# Autodesk Inventor assembly: ASY PRS 2 Filter column D1200
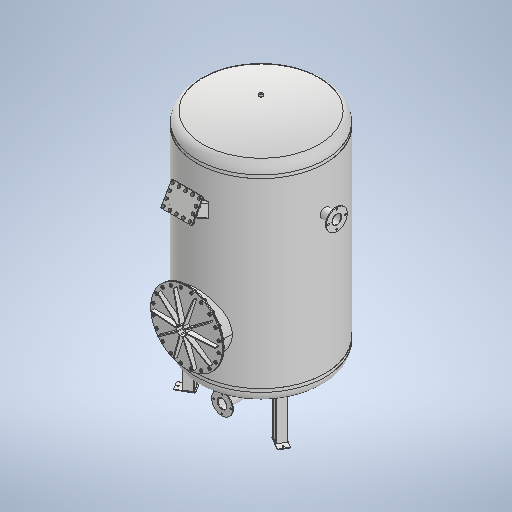
[picture p0: Inventor's stored thumbnail of the model, 512x512]
Saved by Autodesk Inventor 2026.2 (Build 302298000, 298)
## iProperties
Created: 2025-02-13
Part Number: ASY PRS 2 Filter column D1200
Document SubType Name: Assembly
Designer: admin
Mass: 296006 g
Surface Area: 199460 cm^2
Volume: 66339.5 cm^3
Density: 4.46198 g/cm^3
Author: pokla
Revision Number: 3
## Documents named in this file (23)
- C:\Users\admin\Documents\Inventor\PRS-Purovsk\ASY PRS 2 Filter column D1200.iam
- C:\Users\admin\Documents\Inventor\PRS-Purovsk\PRS 0101 main shell D1200.ipt
- C:\Users\admin\Documents\Inventor\PRS-Purovsk\PRS 1604 dished head_D1200.ipt
- C:\Users\admin\Documents\Inventor\PRS-Purovsk\Fitting G1_D1200.ipt
- C:\Users\admin\Documents\Inventor\PRS-Purovsk\PRS 1633 charging blind flange_D1200.ipt
- C:\Users\admin\Documents\Inventor\PRS-Purovsk\ASY PRS 1791 top funnel 50-90_1000x90_D1200.iam
- C:\Users\admin\Documents\Inventor\PRS-Purovsk\PRS 8123 pallet jack dummy_D1200.ipt
- C:\Users\admin\Documents\Inventor\PRS-Purovsk\ASY PRS 1610 charging hatch_D1200.iam
- C:\Users\admin\Documents\Inventor\PRS-Purovsk\PRS 9612 accses hatch flangeipt_D1200.ipt
- C:\Users\admin\Documents\Inventor\PRS-Purovsk\PRS 9615 FDS tube 5_D1200.ipt
- C:\Users\admin\Documents\Inventor\PRS-Purovsk\PRS 9612 FDS tube 2_D1200.ipt
- C:\Users\admin\Documents\Inventor\PRS-Purovsk\cc\JIS B 2312 90 Deg Long Elbow Steel 80A x Sch 40.ipt
- C:\Users\admin\Documents\Inventor\PRS-Purovsk\PRS 9311 accses hatch tube_D1200.ipt
- C:\Users\admin\Documents\Inventor\PRS-Purovsk\PRS 9432 FDS free flange DN90_D1200.ipt
- C:\Users\admin\Documents\Inventor\PRS-Purovsk\PRS 9431 FDS flange DN90_D1200.ipt
- C:\Users\admin\Documents\Inventor\PRS-Purovsk\PRS 9614 FDS tube 4_D1200.ipt
- C:\Users\admin\Documents\Inventor\PRS-Purovsk\PRS 9613 FDS tube 3_D1200.ipt
- C:\Users\admin\Documents\Inventor\PRS-Purovsk\ASY PRS 9690 Filter legs D1200.iam
- C:\Users\admin\Documents\Inventor\PRS-Purovsk\ASY PRS 9800 DrainSystemBottom_D1200.iam
- C:\Users\admin\Documents\Inventor\PRS-Purovsk\cc\en-US\ISO 4018\ISO 4018 - M16 x 40.ipt
- C:\Users\admin\Documents\Inventor\PRS-Purovsk\cc\en-US\ISO 7089\ISO 7089 - 16 - 140 HV(1).ipt
- C:\Users\admin\Documents\Inventor\PRS-Purovsk\cc\en-US\ISO 4032(2)\ISO 4032 - M16 - ISO.ipt
- C:\Users\admin\Documents\Inventor\PRS-Purovsk\ASY 9610 charging hatch.iam
## Components (84 placed, 22 different names)
1. PRS 0101 main shell D1200:1 — Flush:2, Rigid:14, Rigid:15, Rigid:16, Flush:4, Mate:1, Mate:3
2. PRS 1604 dished head_D1200:1 — Rigid:15, Mate:5, Rigid:20, Mate:8
3. PRS 1604 dished head_D1200:2 — Rigid:15, Rigid:14, Mate:4
4. Fitting G1_D1200:1 — Rigid:15
5. PRS 1633 charging blind flange_D1200:1 — Rigid:67
6. ASY PRS 1791 top funnel 50-90_1000x90_D1200:1 [sub-assembly] — Rotational:72
7. pallet jack dummy_1200:1
8. PRS 1633 charging blind flange_D1200:2 — Rigid:77
9. PRS 1633 charging blind flange_D1200:3 — Rotational:72, Rigid:78
10. ASY PRS 1610 charging hatch_D1200:1 [sub-assembly] — Rigid:24, Mate:11, Mate:12, Mate:13, Mate:14, Mate:15, Mate:16, Mate:17, Mate:18, Mate:19, Mate:20, Mate:21, Mate:22, Mate:23, Mate:24, Mate:25, Mate:26, Mate:27, Mate:28, Mate:29, Mate:30, Mate:31, Mate:32, Mate:33, Mate:34, Mate:35, Mate:36, Mate:37, Mate:38, Mate:39, Mate:40, Mate:41, Mate:42, Mate:43, Mate:44, Mate:45, Mate:46, Mate:47, Mate:48, Mate:49, Mate:50, Mate:51, Mate:53, Mate:55, Mate:57, Mate:59, Mate:61, Mate:63, Mate:65, Mate:67, Mate:69, Mate:71, Mate:73, Mate:75, Mate:77, Mate:79, Mate:81, Mate:83, Mate:85, Mate:87, Mate:89
11. PRS 9612 accses hatch flangeipt_D1200:1 — Rigid:23, Rigid:24, Mate:52, Mate:54, Mate:56, Mate:58, Mate:60, Mate:62, Mate:64, Mate:66, Mate:68, Mate:70, Mate:72, Mate:74, Mate:76, Mate:78, Mate:80, Mate:82, Mate:84, Mate:86, Mate:88, Mate:90
12. PRS 9615 FDS tube 5_D1200:1 — Rigid:73, Rigid:77, Mate:3
13. PRS 9612 FDS tube 2_D1200:1 — Rigid:62, Rigid:78, Mate:4
14. JIS B 2312 90 Deg Long Elbow Steel 80A x Sch 40:1 — Rigid:62, Rigid:73
15. PRS 9311 accses hatch tube_D1200:1 — Rigid:16, Rigid:23
16. PRS 9432 FDS free flange DN90_D1200:1 — Rigid:76, Rotational:71, Rotational:78
17. PRS 9431 FDS flange DN90_D1200:1 — Rigid:76
18. PRS 9614 FDS tube 4_D1200:1 — Rigid:79, Rotational:71, Rigid:20
19. PRS 9613 FDS tube 3_D1200:1 — Rigid:68, Rigid:67
20. JIS B 2312 90 Deg Long Elbow Steel 80A x Sch 40:2 — Rigid:68, Rigid:79
21. Fitting G1_D1200:2 — Mate:6, Mate:7, Mate:8
22. ASY PRS 9800 DrainSystemBottom_D1200:1 [sub-assembly] — Rotational:78
23. ASY PRS 9690 Filter legs D1200:1 [sub-assembly] — Flush:5, Flush:6, Mate:2
24. ISO 4018 M16 x 40:1 — Mate:11, Mate:12
25. ISO 7089 16:1 — Mate:51, Mate:52, Insert:1
26. ISO 4032 M16:1 — Insert:1
27. ISO 4018 M16 x 40:2 — Mate:13, Mate:14
28. ISO 4018 M16 x 40:3 — Mate:15, Mate:16
29. ISO 4018 M16 x 40:4 — Mate:17, Mate:18
30. ISO 4018 M16 x 40:5 — Mate:19, Mate:20
31. ISO 4018 M16 x 40:6 — Mate:21, Mate:22
32. ISO 4018 M16 x 40:7 — Mate:23, Mate:24
33. ISO 4018 M16 x 40:8 — Mate:25, Mate:26
34. ISO 4018 M16 x 40:9 — Mate:27, Mate:28
35. ISO 4018 M16 x 40:10 — Mate:29, Mate:30
36. ISO 4018 M16 x 40:11 — Mate:31, Mate:32
37. ISO 4018 M16 x 40:12 — Mate:33, Mate:34
38. ISO 4018 M16 x 40:13 — Mate:35, Mate:36
39. ISO 4018 M16 x 40:14 — Mate:37, Mate:38
40. ISO 4018 M16 x 40:15 — Mate:39, Mate:40
41. ISO 4018 M16 x 40:16 — Mate:41, Mate:42
42. ISO 4018 M16 x 40:17 — Mate:43, Mate:44
43. ISO 4018 M16 x 40:18 — Mate:45, Mate:46
44. ISO 4018 M16 x 40:19 — Mate:47, Mate:48
45. ISO 4018 M16 x 40:20 — Mate:49, Mate:50
46. ISO 7089 16:2 — Mate:53, Mate:54, Insert:2
47. ISO 7089 16:3 — Mate:55, Mate:56, Insert:3
48. ISO 7089 16:4 — Mate:57, Mate:58, Insert:4
49. ISO 7089 16:5 — Mate:59, Mate:60, Insert:5
50. ISO 7089 16:6 — Mate:61, Mate:62, Insert:6
51. ISO 7089 16:7 — Mate:63, Mate:64, Insert:7
52. ISO 7089 16:8 — Mate:65, Mate:66, Insert:8
53. ISO 7089 16:9 — Mate:67, Mate:68, Insert:9
54. ISO 7089 16:10 — Mate:69, Mate:70, Insert:10
55. ISO 7089 16:11 — Mate:71, Mate:72, Insert:11
56. ISO 7089 16:12 — Mate:73, Mate:74, Insert:12
57. ISO 7089 16:13 — Mate:75, Mate:76, Insert:13
58. ISO 7089 16:14 — Mate:77, Mate:78, Insert:14
59. ISO 7089 16:15 — Mate:79, Mate:80, Insert:15
60. ISO 7089 16:16 — Mate:81, Mate:82, Insert:16
61. ISO 7089 16:17 — Mate:83, Mate:84, Insert:17
62. ISO 7089 16:18 — Mate:85, Mate:86, Insert:18
63. ISO 7089 16:19 — Mate:87, Mate:88, Insert:19
64. ISO 7089 16:20 — Mate:89, Mate:90, Insert:20
65. ISO 4032 M16:2 — Insert:2
66. ISO 4032 M16:3 — Insert:3
67. ISO 4032 M16:4 — Insert:4
68. ISO 4032 M16:5 — Insert:5
69. ISO 4032 M16:6 — Insert:6
70. ISO 4032 M16:7 — Insert:7
71. ISO 4032 M16:8 — Insert:8
72. ISO 4032 M16:9 — Insert:9
73. ISO 4032 M16:10 — Insert:10
74. ISO 4032 M16:11 — Insert:11
75. ISO 4032 M16:12 — Insert:12
76. ISO 4032 M16:13 — Insert:13
77. ISO 4032 M16:14 — Insert:14
78. ISO 4032 M16:15 — Insert:15
79. ISO 4032 M16:16 — Insert:16
80. ISO 4032 M16:17 — Insert:17
81. ISO 4032 M16:18 — Insert:18
82. ISO 4032 M16:19 — Insert:19
83. ISO 4032 M16:20 — Insert:20
84. ASY 9610 charging hatch:1 [sub-assembly]
## Relationships (133: Mate 90, Insert 20, WeldJoint 15, Flush 4, RevoluteJoint 3, Tangent 1)
- Rigid:15 [WeldJoint]: PRS 1604 dished head_D1200:2 ↔ Fitting G1_D1200:1
- Rigid:62 [WeldJoint]: PRS 9612 FDS tube 2_D1200:1 ↔ JIS B 2312 90 Deg Long Elbow Steel 80A x Sch 40:1
- Rigid:68 [WeldJoint]: PRS 9613 FDS tube 3_D1200:1 ↔ JIS B 2312 90 Deg Long Elbow Steel 80A x Sch 40:2
- Rigid:67 [WeldJoint]: PRS 1633 charging blind flange_D1200:1 ↔ PRS 9613 FDS tube 3_D1200:1
- Rigid:79 [WeldJoint]: PRS 9614 FDS tube 4_D1200:1 ↔ JIS B 2312 90 Deg Long Elbow Steel 80A x Sch 40:2
- Rigid:73 [WeldJoint]: PRS 9615 FDS tube 5_D1200:1 ↔ JIS B 2312 90 Deg Long Elbow Steel 80A x Sch 40:1
- Rigid:76 [WeldJoint]: PRS 9432 FDS free flange DN90_D1200:1 ↔ PRS 9431 FDS flange DN90_D1200:1
- Rotational:71 [RevoluteJoint]: PRS 9432 FDS free flange DN90_D1200:1 ↔ PRS 9614 FDS tube 4_D1200:1
- Rigid:77 [WeldJoint]: PRS 1633 charging blind flange_D1200:2 ↔ PRS 9615 FDS tube 5_D1200:1
- Rotational:72 [RevoluteJoint]: ASY PRS 1791 top funnel 50-90_1000x90_D1200:1 ↔ PRS 1633 charging blind flange_D1200:3
- Rigid:78 [WeldJoint]: PRS 1633 charging blind flange_D1200:3 ↔ PRS 9612 FDS tube 2_D1200:1
- Rotational:78 [RevoluteJoint]: PRS 9432 FDS free flange DN90_D1200:1 ↔ ASY PRS 9800 DrainSystemBottom_D1200:1
- Flush:2: PRS 0101 main shell D1200:1
- Rigid:14 [WeldJoint]: PRS 0101 main shell D1200:1 ↔ PRS 1604 dished head_D1200:2
- Rigid:15 [WeldJoint]: PRS 0101 main shell D1200:1 ↔ PRS 1604 dished head_D1200:1
- Rigid:16 [WeldJoint] (20 mm): PRS 0101 main shell D1200:1 ↔ PRS 9311 accses hatch tube_D1200:1
- Flush:4: PRS 0101 main shell D1200:1
- Mate:1: PRS 0101 main shell D1200:1
- Flush:5: ASY PRS 9690 Filter legs D1200:1
- Flush:6: ASY PRS 9690 Filter legs D1200:1
- Mate:2: ASY PRS 9690 Filter legs D1200:1
- Mate:3: PRS 0101 main shell D1200:1 ↔ PRS 9615 FDS tube 5_D1200:1
- Mate:4: PRS 1604 dished head_D1200:2 ↔ PRS 9612 FDS tube 2_D1200:1
- Mate:5 (300 mm): PRS 1604 dished head_D1200:1
- Rigid:20 [WeldJoint]: PRS 1604 dished head_D1200:1 ↔ PRS 9614 FDS tube 4_D1200:1
- Mate:6: Fitting G1_D1200:2
- Mate:7 (150 mm): Fitting G1_D1200:2
- Mate:8: PRS 1604 dished head_D1200:1 ↔ Fitting G1_D1200:2
- [Mate]: PRS 0101 main shell D1200:1 ↔ ASY 9610 charging hatch:1
- [Mate]: PRS 0101 main shell D1200:1 ↔ ASY 9610 charging hatch:1
- Rigid:23 [WeldJoint]: PRS 9612 accses hatch flangeipt_D1200:1 ↔ PRS 9311 accses hatch tube_D1200:1
- Rigid:24 [WeldJoint]: ASY PRS 1610 charging hatch_D1200:1 ↔ PRS 9612 accses hatch flangeipt_D1200:1
- [Tangent] (80 mm): PRS 0101 main shell D1200:1 ↔ ASY 9610 charging hatch:1
- Mate:11: ASY PRS 1610 charging hatch_D1200:1 ↔ ISO 4018 M16 x 40:1
- Mate:12: ASY PRS 1610 charging hatch_D1200:1 ↔ ISO 4018 M16 x 40:1
- Mate:13: ASY PRS 1610 charging hatch_D1200:1 ↔ ISO 4018 M16 x 40:2
- Mate:14: ASY PRS 1610 charging hatch_D1200:1 ↔ ISO 4018 M16 x 40:2
- Mate:15: ASY PRS 1610 charging hatch_D1200:1 ↔ ISO 4018 M16 x 40:3
- Mate:16: ASY PRS 1610 charging hatch_D1200:1 ↔ ISO 4018 M16 x 40:3
- Mate:17: ASY PRS 1610 charging hatch_D1200:1 ↔ ISO 4018 M16 x 40:4
- Mate:18: ASY PRS 1610 charging hatch_D1200:1 ↔ ISO 4018 M16 x 40:4
- Mate:19: ASY PRS 1610 charging hatch_D1200:1 ↔ ISO 4018 M16 x 40:5
- Mate:20: ASY PRS 1610 charging hatch_D1200:1 ↔ ISO 4018 M16 x 40:5
- Mate:21: ASY PRS 1610 charging hatch_D1200:1 ↔ ISO 4018 M16 x 40:6
- Mate:22: ASY PRS 1610 charging hatch_D1200:1 ↔ ISO 4018 M16 x 40:6
- Mate:23: ASY PRS 1610 charging hatch_D1200:1 ↔ ISO 4018 M16 x 40:7
- Mate:24: ASY PRS 1610 charging hatch_D1200:1 ↔ ISO 4018 M16 x 40:7
- Mate:25: ASY PRS 1610 charging hatch_D1200:1 ↔ ISO 4018 M16 x 40:8
- Mate:26: ASY PRS 1610 charging hatch_D1200:1 ↔ ISO 4018 M16 x 40:8
- Mate:27: ASY PRS 1610 charging hatch_D1200:1 ↔ ISO 4018 M16 x 40:9
- Mate:28: ASY PRS 1610 charging hatch_D1200:1 ↔ ISO 4018 M16 x 40:9
- Mate:29: ASY PRS 1610 charging hatch_D1200:1 ↔ ISO 4018 M16 x 40:10
- Mate:30: ASY PRS 1610 charging hatch_D1200:1 ↔ ISO 4018 M16 x 40:10
- Mate:31: ASY PRS 1610 charging hatch_D1200:1 ↔ ISO 4018 M16 x 40:11
- Mate:32: ASY PRS 1610 charging hatch_D1200:1 ↔ ISO 4018 M16 x 40:11
- Mate:33: ASY PRS 1610 charging hatch_D1200:1 ↔ ISO 4018 M16 x 40:12
- Mate:34: ASY PRS 1610 charging hatch_D1200:1 ↔ ISO 4018 M16 x 40:12
- Mate:35: ASY PRS 1610 charging hatch_D1200:1 ↔ ISO 4018 M16 x 40:13
- Mate:36: ASY PRS 1610 charging hatch_D1200:1 ↔ ISO 4018 M16 x 40:13
- Mate:37: ASY PRS 1610 charging hatch_D1200:1 ↔ ISO 4018 M16 x 40:14
- Mate:38: ASY PRS 1610 charging hatch_D1200:1 ↔ ISO 4018 M16 x 40:14
- Mate:39: ASY PRS 1610 charging hatch_D1200:1 ↔ ISO 4018 M16 x 40:15
- Mate:40: ASY PRS 1610 charging hatch_D1200:1 ↔ ISO 4018 M16 x 40:15
- Mate:41: ASY PRS 1610 charging hatch_D1200:1 ↔ ISO 4018 M16 x 40:16
- Mate:42: ASY PRS 1610 charging hatch_D1200:1 ↔ ISO 4018 M16 x 40:16
- Mate:43: ASY PRS 1610 charging hatch_D1200:1 ↔ ISO 4018 M16 x 40:17
- Mate:44: ASY PRS 1610 charging hatch_D1200:1 ↔ ISO 4018 M16 x 40:17
- Mate:45: ASY PRS 1610 charging hatch_D1200:1 ↔ ISO 4018 M16 x 40:18
- Mate:46: ASY PRS 1610 charging hatch_D1200:1 ↔ ISO 4018 M16 x 40:18
- Mate:47: ASY PRS 1610 charging hatch_D1200:1 ↔ ISO 4018 M16 x 40:19
- Mate:48: ASY PRS 1610 charging hatch_D1200:1 ↔ ISO 4018 M16 x 40:19
- Mate:49: ASY PRS 1610 charging hatch_D1200:1 ↔ ISO 4018 M16 x 40:20
- Mate:50: ASY PRS 1610 charging hatch_D1200:1 ↔ ISO 4018 M16 x 40:20
- Mate:51: ASY PRS 1610 charging hatch_D1200:1 ↔ ISO 7089 16:1
- Mate:52: PRS 9612 accses hatch flangeipt_D1200:1 ↔ ISO 7089 16:1
- Mate:53: ASY PRS 1610 charging hatch_D1200:1 ↔ ISO 7089 16:2
- Mate:54: PRS 9612 accses hatch flangeipt_D1200:1 ↔ ISO 7089 16:2
- Mate:55: ASY PRS 1610 charging hatch_D1200:1 ↔ ISO 7089 16:3
- Mate:56: PRS 9612 accses hatch flangeipt_D1200:1 ↔ ISO 7089 16:3
- Mate:57: ASY PRS 1610 charging hatch_D1200:1 ↔ ISO 7089 16:4
- Mate:58: PRS 9612 accses hatch flangeipt_D1200:1 ↔ ISO 7089 16:4
- Mate:59: ASY PRS 1610 charging hatch_D1200:1 ↔ ISO 7089 16:5
- Mate:60: PRS 9612 accses hatch flangeipt_D1200:1 ↔ ISO 7089 16:5
- Mate:61: ASY PRS 1610 charging hatch_D1200:1 ↔ ISO 7089 16:6
- Mate:62: PRS 9612 accses hatch flangeipt_D1200:1 ↔ ISO 7089 16:6
- Mate:63: ASY PRS 1610 charging hatch_D1200:1 ↔ ISO 7089 16:7
- Mate:64: PRS 9612 accses hatch flangeipt_D1200:1 ↔ ISO 7089 16:7
- Mate:65: ASY PRS 1610 charging hatch_D1200:1 ↔ ISO 7089 16:8
- Mate:66: PRS 9612 accses hatch flangeipt_D1200:1 ↔ ISO 7089 16:8
- Mate:67: ASY PRS 1610 charging hatch_D1200:1 ↔ ISO 7089 16:9
- Mate:68: PRS 9612 accses hatch flangeipt_D1200:1 ↔ ISO 7089 16:9
- Mate:69: ASY PRS 1610 charging hatch_D1200:1 ↔ ISO 7089 16:10
- Mate:70: PRS 9612 accses hatch flangeipt_D1200:1 ↔ ISO 7089 16:10
- Mate:71: ASY PRS 1610 charging hatch_D1200:1 ↔ ISO 7089 16:11
- Mate:72: PRS 9612 accses hatch flangeipt_D1200:1 ↔ ISO 7089 16:11
- Mate:73: ASY PRS 1610 charging hatch_D1200:1 ↔ ISO 7089 16:12
- Mate:74: PRS 9612 accses hatch flangeipt_D1200:1 ↔ ISO 7089 16:12
- Mate:75: ASY PRS 1610 charging hatch_D1200:1 ↔ ISO 7089 16:13
- Mate:76: PRS 9612 accses hatch flangeipt_D1200:1 ↔ ISO 7089 16:13
- Mate:77: ASY PRS 1610 charging hatch_D1200:1 ↔ ISO 7089 16:14
- Mate:78: PRS 9612 accses hatch flangeipt_D1200:1 ↔ ISO 7089 16:14
- Mate:79: ASY PRS 1610 charging hatch_D1200:1 ↔ ISO 7089 16:15
- Mate:80: PRS 9612 accses hatch flangeipt_D1200:1 ↔ ISO 7089 16:15
- Mate:81: ASY PRS 1610 charging hatch_D1200:1 ↔ ISO 7089 16:16
- Mate:82: PRS 9612 accses hatch flangeipt_D1200:1 ↔ ISO 7089 16:16
- Mate:83: ASY PRS 1610 charging hatch_D1200:1 ↔ ISO 7089 16:17
- Mate:84: PRS 9612 accses hatch flangeipt_D1200:1 ↔ ISO 7089 16:17
- Mate:85: ASY PRS 1610 charging hatch_D1200:1 ↔ ISO 7089 16:18
- Mate:86: PRS 9612 accses hatch flangeipt_D1200:1 ↔ ISO 7089 16:18
- Mate:87: ASY PRS 1610 charging hatch_D1200:1 ↔ ISO 7089 16:19
- Mate:88: PRS 9612 accses hatch flangeipt_D1200:1 ↔ ISO 7089 16:19
- Mate:89: ASY PRS 1610 charging hatch_D1200:1 ↔ ISO 7089 16:20
- Mate:90: PRS 9612 accses hatch flangeipt_D1200:1 ↔ ISO 7089 16:20
- Insert:1: ISO 7089 16:1 ↔ ISO 4032 M16:1
- Insert:2: ISO 7089 16:2 ↔ ISO 4032 M16:2
- Insert:3: ISO 7089 16:3 ↔ ISO 4032 M16:3
- Insert:4: ISO 7089 16:4 ↔ ISO 4032 M16:4
- Insert:5: ISO 7089 16:5 ↔ ISO 4032 M16:5
- Insert:6: ISO 7089 16:6 ↔ ISO 4032 M16:6
- Insert:7: ISO 7089 16:7 ↔ ISO 4032 M16:7
- Insert:8: ISO 7089 16:8 ↔ ISO 4032 M16:8
- Insert:9: ISO 7089 16:9 ↔ ISO 4032 M16:9
- Insert:10: ISO 7089 16:10 ↔ ISO 4032 M16:10
- Insert:11: ISO 7089 16:11 ↔ ISO 4032 M16:11
- Insert:12: ISO 7089 16:12 ↔ ISO 4032 M16:12
- Insert:13: ISO 7089 16:13 ↔ ISO 4032 M16:13
- Insert:14: ISO 7089 16:14 ↔ ISO 4032 M16:14
- Insert:15: ISO 7089 16:15 ↔ ISO 4032 M16:15
- Insert:16: ISO 7089 16:16 ↔ ISO 4032 M16:16
- Insert:17: ISO 7089 16:17 ↔ ISO 4032 M16:17
- Insert:18: ISO 7089 16:18 ↔ ISO 4032 M16:18
- Insert:19: ISO 7089 16:19 ↔ ISO 4032 M16:19
- Insert:20: ISO 7089 16:20 ↔ ISO 4032 M16:20
